# Autodesk Inventor assembly: 684AZZ
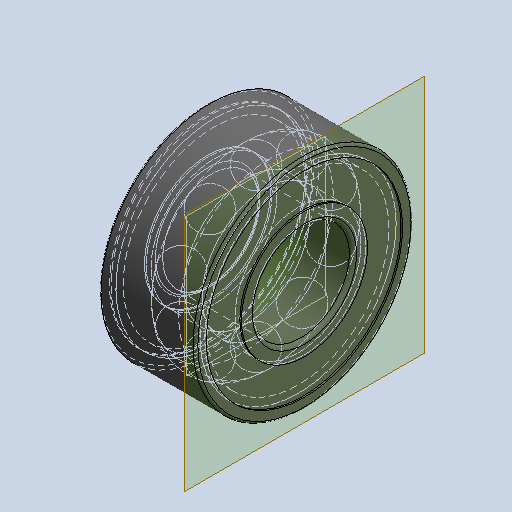
[picture p0: Inventor's stored thumbnail of the model, 512x512]
Saved by Autodesk Inventor 2022 (Build 260153000, 153)
## iProperties
Category: PARTsolutions
Company: NSK_RB
Part Number: 684AZZ
Catalog Web Link: www.cadenas.de
Description: Shielded Type ZZ-ZZS-
Vendor: NSK_RB
Document SubType Name: Assembly
Designer: partserver
Manufacturer: NSK_RB
Mass: 1.01 g
Surface Area: 5.89581 cm^2
Volume: 0.13253 cm^3
Density: 7.62093 g/cm^3
PSOL_IDENT_0: {$CADENAS_DATA\23d-libs\nsk_rb\roller_bearings\deep_groove_bb\exstra_small_miniatur_bb\metric_design
PSOL_IDENT_1: \shielded_type_zz_zzs_asmtab.prj},172 {VTYP=3D},{STYP=ASSTAB},{NB=684AZZ},{LINA=684AZZ},{NN=Shielded
PSOL_IDENT_2: Type ZZ-ZZS},{DATE=30.03.2022 01:55:07},{GEOMDATE=14.01.2008},{VERSION=},{LINEID=220},{WBVAR=},{WBN
PSOL_IDENT_3: UMERIC=}  {NB=684AZZ},{LINA=684AZZ},{KT=DUMMY},{IDNR=},{STAN=Standard},{ORDER=684AZZ},{SD=4.0},{X=4.
PSOL_IDENT_4: 0},{DI1=5.20},{DI2=5.20},{SDE1=7.50},{SDE2=8.10},{D=9},{DD=9},{B=0.0},{B1=4.0},{R=0.00},{R1=0.15},{C
PSOL_IDENT_5: R1=640},{COR1=225},{CR2=65},{COR2=23.0},{LG=53000},{LO=63000},{DA=0.0},{DB=5.2},{DA1=0.0},{DB1=8.1},
PSOL_IDENT_6: {RA=0.00},{RB=0.10},{MASS=1.01},{SC=1},{PPATH=shielded_type_zz_zzs_asmtpl.prj}
NB: 684AZZ
NN: Shielded Type ZZ-ZZS
NBSYN: $ORDER.
LINA: 684AZZ
CATALOG: NSK Rolling Bearing
STAN: Standard
ORDER: 684AZZ
SD: 4
D: 9
B1: 4
R1: 0.15
CR1: 640
COR1: 225
CR2: 65
COR2: 23
LG: 53000
DB: 5.2
DB1: 8.1
RB: 0.1
MASS: 1.01
SUPPLIER: NSK_RB
ARTICLENO: 684AZZ
BOMINFO: 684AZZ
CREATOR: CADENAS GmbH
Title: 684AZZ
Author: Cadenas PARTsolutions
## Documents named in this file (6)
- C:\Users\micha\Desktop\Rat Basketball 3D Files\Hoop assembly\684AZZ.iam
- C:\Users\micha\Desktop\Rat Basketball 3D Files\Hoop assembly\Completed Hoop\NSK_RB_684AZZ\AIS2022\684AZZ Outer Ring.ipt
- C:\Users\micha\Desktop\Rat Basketball 3D Files\Hoop assembly\Completed Hoop\NSK_RB_684AZZ\AIS2022\684AZZ Inner Ring.ipt
- C:\Users\micha\Desktop\Rat Basketball 3D Files\Hoop assembly\Completed Hoop\NSK_RB_684AZZ\AIS2022\684AZZ Shield1.ipt
- C:\Users\micha\Desktop\Rat Basketball 3D Files\Hoop assembly\Completed Hoop\NSK_RB_684AZZ\AIS2022\684AZZ Ball.ipt
- C:\Users\micha\Desktop\Rat Basketball 3D Files\Hoop assembly\Completed Hoop\NSK_RB_684AZZ\AIS2022\684AZZ Shield2.ipt
## Components (14 placed, 5 different names)
1. 684AZZ Outer Ring:1
2. 684AZZ Inner Ring:1 — Symmetry:1
3. 684AZZ Shield1:1
4. 684AZZ Ball:1
5. 684AZZ Ball:2
6. 684AZZ Ball:3
7. 684AZZ Ball:4
8. 684AZZ Ball:5
9. 684AZZ Ball:6
10. 684AZZ Ball:7
11. 684AZZ Ball:8
12. 684AZZ Ball:9
13. 684AZZ Ball:10
14. 684AZZ Shield2:1
## Relationships (1: Symmetry 1)
- Symmetry:1: 684AZZ Inner Ring:1
